# Autodesk Inventor assembly: MMBOT
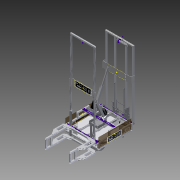
[picture p0: Inventor's stored thumbnail of the model, 180x180]
Saved by Autodesk Inventor 2013 (Build 170138000, 138)
## iProperties
Created: 2015-01-16
Part Number: MMBOT
Document SubType Name: Assembly
Designer: Randall
Translation Standard: STEP AP214IS
FileName: C:\Users\eedoga.OHSD\Desktop\MMBOT.stp
PreProcessor: Autodesk Inventor 2013
PostProcessor: Build: 138, Release: 2013 RTM - Date: Thu 03/01/2012
Sent Units: inch
Uncertainty: 0.00039370078740199997
Author: Randall
## Documents named in this file (42)
- C:\inventor #2\MMLifter\Workspaces\Workspace\MMBOT.iam
- C:\inventor #2\MMLifter\Workspaces\Workspace\Cchannel27inch.ipt
- C:\inventor #2\MMLifter\Workspaces\Workspace\Chassis_Channel_26_AndyMark_am-0202.ipt
- C:\inventor #2\MMLifter\Workspaces\Workspace\Chassis_CornerConnect_AndyMark_am-0212.ipt
- C:\inventor #2\MMLifter\Workspaces\Workspace\HolonomicCornerBracket.ipt
- C:\inventor #2\MMLifter\Workspaces\Workspace\HolonomicCornerBracket02.ipt
- C:\inventor #2\MMLifter\Workspaces\Workspace\Toughbox-nano-500-key-long-asm.iam
- C:\inventor #2\MMLifter\Workspaces\Workspace\8-Molded-Trick-Wheel.iam
- C:\inventor #2\MMLifter\Workspaces\Workspace\HolonomicCornerBracket_MIR.ipt
- C:\inventor #2\MMLifter\Workspaces\Workspace\HolonomicCornerBracket02_MIR.ipt
- C:\inventor #2\MMLifter\Workspaces\Workspace\Toughbox-nano-500-key-long-asm_MIR.iam
- C:\inventor #2\MMLifter\Workspaces\Workspace\8-Molded-Trick-Wheel_MIR.iam
- C:\inventor #2\MMLifter\Workspaces\Workspace\HolonomicCornerBracket_MIR1.ipt
- C:\inventor #2\MMLifter\Workspaces\Workspace\HolonomicCornerBracket02_MIR1.ipt
- C:\inventor #2\MMLifter\Workspaces\Workspace\Toughbox-nano-500-key-long-asm_MIR1.iam
- C:\inventor #2\MMLifter\Workspaces\Workspace\8-Molded-Trick-Wheel_MIR1.iam
- C:\inventor #2\MMLifter\Workspaces\Workspace\HolonomicCornerBracket_MIR_MIR.ipt
- C:\inventor #2\MMLifter\Workspaces\Workspace\HolonomicCornerBracket02_MIR_MIR.ipt
- C:\inventor #2\MMLifter\Workspaces\Workspace\Toughbox-nano-500-key-long-asm_MIR_MIR.iam
- C:\inventor #2\MMLifter\Workspaces\Workspace\8-Molded-Trick-Wheel_MIR_MIR.iam
- C:\inventor #2\MMLifter\Workspaces\Workspace\3inchUp.ipt
- C:\inventor #2\MMLifter\Workspaces\Workspace\SideLong.ipt
- C:\inventor #2\MMLifter\Workspaces\Workspace\backlong.ipt
- C:\inventor #2\MMLifter\Workspaces\Workspace\channelBracket02.ipt
- C:\inventor #2\MMLifter\Workspaces\Workspace\8020-1010 54upthingy.ipt
- C:\inventor #2\MMLifter\Workspaces\Workspace\6715.iam
- C:\inventor #2\MMLifter\Workspaces\Workspace\MMMainLiftTopCrossBar.ipt
- C:\inventor #2\MMLifter\Workspaces\Workspace\DARTActuator12.iam
- C:\inventor #2\MMLifter\Workspaces\Workspace\mmCenterTowerCross01.ipt
- C:\inventor #2\MMLifter\Workspaces\Workspace\batassj115.iam
- C:\inventor #2\MMLifter\Workspaces\Workspace\Electronics Base.ipt
- C:\inventor #2\MMLifter\Workspaces\Workspace\Battery mechanism motor assembly.iam
- C:\inventor #2\MMLifter\Workspaces\Workspace\RandalLiftMech.iam
- C:\inventor #2\MMLifter\Workspaces\Workspace\PullySystemSmall.iam
- C:\inventor #2\MMLifter\Workspaces\Workspace\dartmount.ipt
- C:\inventor #2\MMLifter\Workspaces\Workspace\armmount01.ipt
- C:\inventor #2\MMLifter\Workspaces\Workspace\gripperAss.iam
- C:\inventor #2\MMLifter\Workspaces\Workspace\SPONSORS BOARD.ipt
- C:\inventor #2\MMLifter\Workspaces\Workspace\liftmechdropper.ipt
- C:\inventor #2\MMLifter\Workspaces\Workspace\The c channel of hinges.ipt
- C:\inventor #2\MMLifter\Workspaces\Workspace\Rear SPONSORS BOARD.0001.ipt
- C:\inventor #2\MMLifter\Workspaces\Workspace\Back sponsors board.ipt
## Components (70 placed, 41 different names)
1. Cchannel27inch:1 — Mate:53, Mate:54
2. Cchannel27inch:2 — Mate:49, Mate:50
3. Chassis_Channel_26_AndyMark_am-0202:1 — Mate:51, Mate:52
4. Chassis_Channel_26_AndyMark_am-0202:2 — Mate:1, Mate:48
5. Chassis_CornerConnect_AndyMark_am-0212:1
6. Chassis_CornerConnect_AndyMark_am-0212:2
7. Chassis_CornerConnect_AndyMark_am-0212:3
8. Chassis_CornerConnect_AndyMark_am-0212:4
9. HolonomicCornerBracket:1 — Mate:1, Mate:2, Mate:3, Mate:152
10. HolonomicCornerBracket02:1
11. Toughbox-nano-500-key-long-asm:1 [sub-assembly] — Mate:151
12. 8-Molded-Trick-Wheel:1 [sub-assembly] — Mate:151, Mate:152
13. HolonomicCornerBracket_MIR:1 — Mate:32, Mate:33, Mate:51, Mate:53, Mate:54, Mate:154
14. HolonomicCornerBracket02_MIR:1
15. Toughbox-nano-500-key-long-asm_MIR:1 [sub-assembly] — Mate:153
16. 8-Molded-Trick-Wheel_MIR:1 [sub-assembly] — Mate:153, Mate:154
17. HolonomicCornerBracket_MIR1:1 — Mate:35, Mate:36, Mate:48, Mate:49, Mate:158
18. HolonomicCornerBracket02_MIR1:1
19. Toughbox-nano-500-key-long-asm_MIR1:1 [sub-assembly] — Mate:157
20. 8-Molded-Trick-Wheel_MIR1:1 [sub-assembly] — Mate:157, Mate:158
21. HolonomicCornerBracket_MIR_MIR:1 — Mate:15, Mate:16, Mate:17, Mate:34, Mate:37, Mate:50, Mate:52, Mate:156
22. HolonomicCornerBracket02_MIR_MIR:1
23. Toughbox-nano-500-key-long-asm_MIR_MIR:1 [sub-assembly] — Mate:155
24. 8-Molded-Trick-Wheel_MIR_MIR:1 [sub-assembly] — Mate:155, Mate:156
25. 3inchUp:1 — Mate:20, Mate:21, Mate:22, Mate:32, Mate:33, Flush:31
26. 3inchUp:2 — Mate:2, Mate:3, Mate:4, Mate:5, Flush:29
27. 3inchUp:3 — Mate:8, Mate:9, Mate:35, Mate:36
28. 3inchUp:4 — Mate:11, Mate:14, Mate:15, Mate:16, Mate:17, Mate:18, Mate:34, Mate:37
29. SideLong:1 — Mate:11, Flush:5, Mate:12, Mate:13, Mate:14, Mate:18, Mate:19, Mate:20, Mate:21, Mate:22, Mate:23, Mate:24, Flush:6, Flush:13, Flush:25, Mate:122
30. SideLong:2 — Mate:4, Mate:5, Mate:6, Mate:7, Flush:1, Mate:8, Mate:9, Mate:10, Flush:4, Flush:12, Flush:18, Mate:143, Mate:146
31. backlong:1 — Mate:10, Flush:4, Flush:5, Mate:12, Mate:13, Flush:16, Mate:109, Mate:110, Mate:111, Mate:112
32. backlong:2 — Mate:6, Mate:7, Mate:19, Mate:23, Mate:24, Mate:73, Mate:74, Flush:14, Flush:15, Flush:17, Mate:77
33. channelBracket02:1 — Mate:70, Mate:71, Mate:73, Flush:13, Mate:75, Flush:15
34. channelBracket02:2 — Mate:55, Mate:72, Mate:74, Flush:12, Mate:76, Flush:14, Mate:78
35. 8020-1010 54upthingy:1 — Mate:55, Mate:68, Mate:69, Mate:76, Mate:79
36. 8020-1010 54upthingy:2 — Mate:70, Mate:75, Flush:19
37. 6715:1 [sub-assembly] — Mate:64, Mate:92, Mate:93
38. 6715:2 [sub-assembly] — Mate:89, Mate:90, Mate:91
39. 6715:3 [sub-assembly] — Mate:56, Mate:60, Mate:61, Mate:62, Mate:63, Mate:68, Mate:69
40. 6715:4 [sub-assembly] — Mate:57, Mate:59
41. MMMainLiftTopCrossBar:1 — Mate:71, Mate:72, Mate:78, Flush:19, Mate:79, Mate:133, Mate:134, Mate:135, Mate:136, Mate:137, Flush:27
42. DARTActuator12:1 [sub-assembly] — Mate:125, Mate:126
43. DARTActuator12:2 [sub-assembly] — Mate:129, Mate:130
44. 3inchUp:5 — Flush:6, Mate:25, Mate:122, Mate:123, Mate:140
45. 3inchUp:6 — Mate:26, Mate:27
46. 3inchUp:7 — Flush:3, Mate:145, Mate:146
47. 3inchUp:8 — Flush:1, Flush:2, Mate:141, Mate:143, Mate:144
48. mmCenterTowerCross01:1 — Flush:2, Flush:3, Mate:124, Flush:26, Mate:138, Flush:28, Mate:141, Mate:144, Mate:145
49. mmCenterTowerCross01:2 — Mate:25, Mate:26, Mate:27, Mate:28, Flush:7, Mate:121, Mate:123, Mate:139, Flush:30, Mate:140
50. batassj115:1 [sub-assembly] — Flush:16, Flush:17, Mate:77, Flush:18
51. Electronics Base:1
52. Battery mechanism motor assembly:1 [sub-assembly]
53. RandalLiftMech:1 [sub-assembly] — Flush:20, Flush:21, Mate:104, Mate:105, Mate:108, Mate:117, Mate:118, Mate:119, Mate:120, Mate:142, Flush:32, Flush:33
54. backlong:3 — Mate:28, Flush:7, Mate:80, Mate:121, Mate:124, Mate:128, Mate:131, Flush:26, Mate:132, Mate:149, Mate:150
55. PullySystemSmall:1 [sub-assembly] — Mate:133, Mate:134, Mate:135
56. dartmount:1 — Mate:80, Mate:125, Mate:126, Mate:131, Mate:149
57. dartmount:2 — Mate:128, Mate:129, Mate:130, Mate:132, Mate:150
58. armmount01:1 — Flush:8, Flush:9, Mate:56, Mate:60, Mate:61, Mate:62, Mate:63, Mate:64, Mate:67, Mate:92, Mate:93
59. armmount01:2 — Mate:57, Mate:59, Flush:10, Flush:11, Mate:66, Mate:89, Mate:90, Mate:91
60. gripperAss:1 [sub-assembly] — Flush:8, Flush:9, Flush:10, Flush:11, Mate:66, Mate:67
61. SPONSORS BOARD:1 — Mate:139, Flush:30, Flush:31
62. SPONSORS BOARD:2 — Mate:138, Flush:28, Flush:29
63. liftmechdropper:1 — Flush:20, Mate:102, Mate:103, Flush:24, Mate:115, Mate:116
64. liftmechdropper:2 — Flush:21, Mate:106, Mate:107, Flush:23, Mate:113, Mate:114
65. The c channel of hinges:1 — Mate:102, Mate:103, Mate:104, Mate:105, Flush:24, Mate:117, Mate:118
66. The c channel of hinges:2 — Mate:106, Mate:107, Mate:108, Flush:23, Mate:119, Mate:120
67. channelBracket02:4 — Mate:109, Mate:111, Mate:113, Mate:114, Flush:25
68. channelBracket02:5 — Mate:110, Mate:112, Mate:115, Mate:116
69. Rear SPONSORS BOARD.0001:1 — Mate:136, Mate:137, Flush:27
70. Back sponsors board:1 — Mate:142, Flush:32, Flush:33
## Relationships (156: Mate 124, Flush 32)
- Mate:1: Chassis_Channel_26_AndyMark_am-0202:2 ↔ HolonomicCornerBracket:1
- Mate:2: HolonomicCornerBracket:1 ↔ 3inchUp:2
- Mate:3: HolonomicCornerBracket:1 ↔ 3inchUp:2
- Mate:4: 3inchUp:2 ↔ SideLong:2
- Mate:5: 3inchUp:2 ↔ SideLong:2
- Mate:6: SideLong:2 ↔ backlong:2
- Mate:7: SideLong:2 ↔ backlong:2
- Flush:1 (228.6 mm): SideLong:2 ↔ 3inchUp:8
- Flush:2: 3inchUp:8 ↔ mmCenterTowerCross01:1
- Flush:3: 3inchUp:7 ↔ mmCenterTowerCross01:1
- Mate:8: 3inchUp:3 ↔ SideLong:2
- Mate:9: 3inchUp:3 ↔ SideLong:2
- Mate:10: SideLong:2 ↔ backlong:1
- Mate:11: 3inchUp:4 ↔ SideLong:1
- Flush:4: SideLong:2 ↔ backlong:1
- Flush:5: SideLong:1 ↔ backlong:1
- Mate:12: SideLong:1 ↔ backlong:1
- Mate:13: SideLong:1 ↔ backlong:1
- Mate:14: 3inchUp:4 ↔ SideLong:1
- Mate:15: HolonomicCornerBracket_MIR_MIR:1 ↔ 3inchUp:4
- Mate:16: HolonomicCornerBracket_MIR_MIR:1 ↔ 3inchUp:4
- Mate:17: HolonomicCornerBracket_MIR_MIR:1 ↔ 3inchUp:4
- Mate:18: 3inchUp:4 ↔ SideLong:1
- Mate:19: SideLong:1 ↔ backlong:2
- Mate:20: 3inchUp:1 ↔ SideLong:1
- Mate:21: 3inchUp:1 ↔ SideLong:1
- Mate:22: 3inchUp:1 ↔ SideLong:1
- Mate:23: SideLong:1 ↔ backlong:2
- Mate:24: SideLong:1 ↔ backlong:2
- Flush:6 (228.6 mm): SideLong:1 ↔ 3inchUp:5
- Mate:25: 3inchUp:5 ↔ mmCenterTowerCross01:2
- Mate:26: 3inchUp:6 ↔ mmCenterTowerCross01:2
- Mate:27: 3inchUp:6 ↔ mmCenterTowerCross01:2
- Mate:28: mmCenterTowerCross01:2 ↔ backlong:3
- Flush:7 (114.3 mm): mmCenterTowerCross01:2 ↔ backlong:3
- Mate:32: HolonomicCornerBracket_MIR:1 ↔ 3inchUp:1
- Mate:33: HolonomicCornerBracket_MIR:1 ↔ 3inchUp:1
- Mate:34: HolonomicCornerBracket_MIR_MIR:1 ↔ 3inchUp:4
- Mate:35: HolonomicCornerBracket_MIR1:1 ↔ 3inchUp:3
- Mate:36: HolonomicCornerBracket_MIR1:1 ↔ 3inchUp:3
- Mate:37: HolonomicCornerBracket_MIR_MIR:1 ↔ 3inchUp:4
- Mate:48: Chassis_Channel_26_AndyMark_am-0202:2 ↔ HolonomicCornerBracket_MIR1:1
- Mate:49: Cchannel27inch:2 ↔ HolonomicCornerBracket_MIR1:1
- Mate:50: Cchannel27inch:2 ↔ HolonomicCornerBracket_MIR_MIR:1
- Mate:51: Chassis_Channel_26_AndyMark_am-0202:1 ↔ HolonomicCornerBracket_MIR:1
- Mate:52: Chassis_Channel_26_AndyMark_am-0202:1 ↔ HolonomicCornerBracket_MIR_MIR:1
- Mate:53: Cchannel27inch:1 ↔ HolonomicCornerBracket_MIR:1
- Mate:54: Cchannel27inch:1 ↔ HolonomicCornerBracket_MIR:1
- Mate:55: channelBracket02:2 ↔ 8020-1010 54upthingy:1
- Flush:8 (91.059 mm): armmount01:1 ↔ gripperAss:1
- Flush:9: armmount01:1 ↔ gripperAss:1
- Mate:56: 6715:3 ↔ armmount01:1
- Mate:57: 6715:4 ↔ armmount01:2
- Mate:59: 6715:4 ↔ armmount01:2
- Mate:60: 6715:3 ↔ armmount01:1
- Mate:61: 6715:3 ↔ armmount01:1
- Mate:62: 6715:3 ↔ armmount01:1
- Mate:63: 6715:3 ↔ armmount01:1
- Mate:64: 6715:1 ↔ armmount01:1
- Flush:10 (65.6336 mm): armmount01:2 ↔ gripperAss:1
- Flush:11: armmount01:2 ↔ gripperAss:1
- Mate:66: armmount01:2 ↔ gripperAss:1
- Mate:67: armmount01:1 ↔ gripperAss:1
- Mate:68: 8020-1010 54upthingy:1 ↔ 6715:3
- Mate:69: 8020-1010 54upthingy:1 ↔ 6715:3
- Mate:70: channelBracket02:1 ↔ 8020-1010 54upthingy:2
- Mate:71: channelBracket02:1 ↔ MMMainLiftTopCrossBar:1
- Mate:72: channelBracket02:2 ↔ MMMainLiftTopCrossBar:1
- Mate:73: backlong:2 ↔ channelBracket02:1
- Mate:74: backlong:2 ↔ channelBracket02:2
- Flush:12 (82.55 mm): SideLong:2 ↔ channelBracket02:2
- Flush:13 (82.55 mm): SideLong:1 ↔ channelBracket02:1
- Mate:75: channelBracket02:1 ↔ 8020-1010 54upthingy:2
- Mate:76: channelBracket02:2 ↔ 8020-1010 54upthingy:1
- Flush:14: backlong:2 ↔ channelBracket02:2
- Flush:15: backlong:2 ↔ channelBracket02:1
- Flush:16: backlong:1 ↔ batassj115:1
- Flush:17: backlong:2 ↔ batassj115:1
- Mate:77: backlong:2 ↔ batassj115:1
- Flush:18 (187.325 mm): SideLong:2 ↔ batassj115:1
- Mate:78: channelBracket02:2 ↔ MMMainLiftTopCrossBar:1
- Flush:19: 8020-1010 54upthingy:2 ↔ MMMainLiftTopCrossBar:1
- Mate:79: 8020-1010 54upthingy:1 ↔ MMMainLiftTopCrossBar:1
- Mate:80: backlong:3 ↔ dartmount:1
- Mate:89: 6715:2 ↔ armmount01:2
- Mate:90: 6715:2 ↔ armmount01:2
- Mate:91: 6715:2 ↔ armmount01:2
- Mate:92: 6715:1 ↔ armmount01:1
- Mate:93: 6715:1 ↔ armmount01:1
- Flush:20: RandalLiftMech:1 ↔ liftmechdropper:1
- Flush:21: RandalLiftMech:1 ↔ liftmechdropper:2
- Mate:102: liftmechdropper:1 ↔ The c channel of hinges:1
- Mate:103: liftmechdropper:1 ↔ The c channel of hinges:1
- Mate:104: RandalLiftMech:1 ↔ The c channel of hinges:1
- Mate:105: RandalLiftMech:1 ↔ The c channel of hinges:1
- Mate:106: liftmechdropper:2 ↔ The c channel of hinges:2
- Mate:107: liftmechdropper:2 ↔ The c channel of hinges:2
- Mate:108: RandalLiftMech:1 ↔ The c channel of hinges:2
- Flush:23: liftmechdropper:2 ↔ The c channel of hinges:2
- Flush:24: liftmechdropper:1 ↔ The c channel of hinges:1
- Mate:109: backlong:1 ↔ channelBracket02:4
- Mate:110: backlong:1 ↔ channelBracket02:5
- Mate:111: backlong:1 ↔ channelBracket02:4
- Mate:112: backlong:1 ↔ channelBracket02:5
- Mate:113: liftmechdropper:2 ↔ channelBracket02:4
- Mate:114: liftmechdropper:2 ↔ channelBracket02:4
- Mate:115: liftmechdropper:1 ↔ channelBracket02:5
- Mate:116: liftmechdropper:1 ↔ channelBracket02:5
- Flush:25 (47.625 mm): SideLong:1 ↔ channelBracket02:4
- Mate:117: RandalLiftMech:1 ↔ The c channel of hinges:1
- Mate:118: RandalLiftMech:1 ↔ The c channel of hinges:1
- Mate:119: RandalLiftMech:1 ↔ The c channel of hinges:2
- Mate:120: RandalLiftMech:1 ↔ The c channel of hinges:2
- Mate:121: mmCenterTowerCross01:2 ↔ backlong:3
- Mate:122: SideLong:1 ↔ 3inchUp:5
- Mate:123: 3inchUp:5 ↔ mmCenterTowerCross01:2
- Mate:124: mmCenterTowerCross01:1 ↔ backlong:3
- Mate:125: DARTActuator12:1 ↔ dartmount:1
- Mate:126 (12.7 mm): DARTActuator12:1 ↔ dartmount:1
- Mate:128: backlong:3 ↔ dartmount:2
- Mate:129: DARTActuator12:2 ↔ dartmount:2
- Mate:130 (12.7 mm): DARTActuator12:2 ↔ dartmount:2
- Mate:131: backlong:3 ↔ dartmount:1
- Flush:26 (114.3 mm): mmCenterTowerCross01:1 ↔ backlong:3
- Mate:132: backlong:3 ↔ dartmount:2
- Mate:133: MMMainLiftTopCrossBar:1 ↔ PullySystemSmall:1
- Mate:134: MMMainLiftTopCrossBar:1 ↔ PullySystemSmall:1
- Mate:135: MMMainLiftTopCrossBar:1 ↔ PullySystemSmall:1
- Mate:136: MMMainLiftTopCrossBar:1 ↔ Rear SPONSORS BOARD.0001:1
- Mate:137: MMMainLiftTopCrossBar:1 ↔ Rear SPONSORS BOARD.0001:1
- Flush:27 (812.8 mm): MMMainLiftTopCrossBar:1 ↔ Rear SPONSORS BOARD.0001:1
- Mate:138: mmCenterTowerCross01:1 ↔ SPONSORS BOARD:2
- Flush:28: mmCenterTowerCross01:1 ↔ SPONSORS BOARD:2
- Flush:29: 3inchUp:2 ↔ SPONSORS BOARD:2
- Mate:139: mmCenterTowerCross01:2 ↔ SPONSORS BOARD:1
- Flush:30: mmCenterTowerCross01:2 ↔ SPONSORS BOARD:1
- Flush:31: 3inchUp:1 ↔ SPONSORS BOARD:1
- Mate:140: 3inchUp:5 ↔ mmCenterTowerCross01:2
- Mate:141: 3inchUp:8 ↔ mmCenterTowerCross01:1
- Mate:142: RandalLiftMech:1 ↔ Back sponsors board:1
- Flush:32 (-533.4 mm): RandalLiftMech:1 ↔ Back sponsors board:1
- Flush:33: RandalLiftMech:1 ↔ Back sponsors board:1
- Mate:143: SideLong:2 ↔ 3inchUp:8
- Mate:144: 3inchUp:8 ↔ mmCenterTowerCross01:1
- Mate:145: 3inchUp:7 ↔ mmCenterTowerCross01:1
- Mate:146: SideLong:2 ↔ 3inchUp:7
- Mate:149: backlong:3 ↔ dartmount:1
- Mate:150: backlong:3 ↔ dartmount:2
- Mate:151: Toughbox-nano-500-key-long-asm:1 ↔ 8-Molded-Trick-Wheel:1
- Mate:152 (12.7 mm): HolonomicCornerBracket:1 ↔ 8-Molded-Trick-Wheel:1
- Mate:153: Toughbox-nano-500-key-long-asm_MIR:1 ↔ 8-Molded-Trick-Wheel_MIR:1
- Mate:154 (12.7 mm): HolonomicCornerBracket_MIR:1 ↔ 8-Molded-Trick-Wheel_MIR:1
- Mate:155: Toughbox-nano-500-key-long-asm_MIR_MIR:1 ↔ 8-Molded-Trick-Wheel_MIR_MIR:1
- Mate:156 (12.7 mm): HolonomicCornerBracket_MIR_MIR:1 ↔ 8-Molded-Trick-Wheel_MIR_MIR:1
- Mate:157: Toughbox-nano-500-key-long-asm_MIR1:1 ↔ 8-Molded-Trick-Wheel_MIR1:1
- Mate:158 (12.7 mm): HolonomicCornerBracket_MIR1:1 ↔ 8-Molded-Trick-Wheel_MIR1:1
